# Autodesk Inventor assembly: Assembly
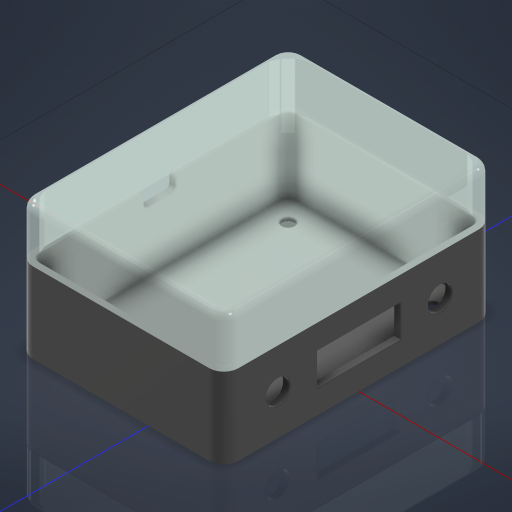
[picture p0: Inventor's stored thumbnail of the model, 512x512]
Saved by Autodesk Inventor 2024 (Build 280153000, 153)
## iProperties
Created: 2023-08-04
Part Number: Assembly
Document SubType Name: Assembly
Designer: Noah
Author: Noah
## Documents named in this file (3)
- N:\Github\love_lamps\inventor\Assembly.iam
- N:\Github\love_lamps\inventor\BaseV2.ipt
- N:\Github\love_lamps\inventor\ShadeV2.ipt
## Components (2 placed, 2 different names)
1. BaseV2:1 — Mate:1, Flush:1, Flush:2
2. ShadeV2:1 — Mate:1, Flush:1, Flush:2
## Relationships (3: Flush 2, Mate 1)
- Mate:1: BaseV2:1 ↔ ShadeV2:1
- Flush:1: BaseV2:1 ↔ ShadeV2:1
- Flush:2: BaseV2:1 ↔ ShadeV2:1
